# Autodesk Inventor assembly: Assembly2
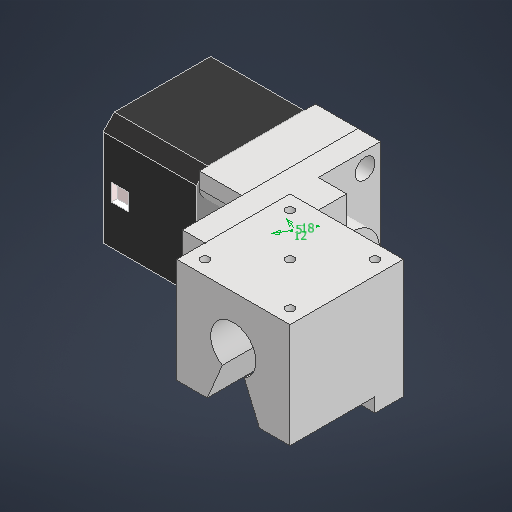
[picture p0: Inventor's stored thumbnail of the model, 512x512]
Saved by Autodesk Inventor 2025.1 (Build 291241000, 241)
## iProperties
Created: 2025-02-02
Part Number: Assembly2
Document SubType Name: Assembly
Designer: jerem
Author: jerem
## Documents named in this file (7)
- C:\Users\jerem\Documents\GitHub\Perovskite-Automated-Synthesis-System\CAD\Gantry\Assembly2.iam
- C:\Users\jerem\Documents\GitHub\Perovskite-Automated-Synthesis-System\CAD\Gantry\X Axis End.ipt
- C:\Users\jerem\Documents\GitHub\Perovskite-Automated-Synthesis-System\CAD\Non 3D Printed Parts\Motors and Servos\NEMA17 Stepper Motor.ipt
- C:\Users\jerem\Documents\GitHub\Perovskite-Automated-Synthesis-System\CAD\Gantry\end motor holder.ipt
- C:\Users\jerem\Documents\GitHub\Perovskite-Automated-Synthesis-System\CAD\Non 3D Printed Parts\Idler.ipt
- C:\Users\jerem\Documents\GitHub\Perovskite-Automated-Synthesis-System\CAD\Non 3D Printed Parts\Rod Coupler.ipt
- C:\Users\jerem\Documents\GitHub\Perovskite-Automated-Synthesis-System\CAD\Gantry\MOTOR standoff.ipt
## Components (6 placed, 6 different names)
1. X Axis End:1 — Flush:1, Mate:13, Mate:14
2. NEMA17 Stepper Motor:1 — Mate:1, Mate:2, Mate:5, Mate:6, Mate:8, Mate:10, Mate:11, Mate:12
3. end motor holder:1 — Mate:1, Mate:2, Flush:1, Mate:13, Mate:14, Mate:15
4. Idler:1 — Mate:5, Mate:6, Mate:9
5. Rod Coupler:1 — Mate:8, Mate:9
6. MOTOR standoff:1 — Mate:10, Mate:11, Mate:12, Mate:15
## Relationships (13: Mate 12, Flush 1)
- Mate:1: NEMA17 Stepper Motor:1 ↔ end motor holder:1
- Mate:2: NEMA17 Stepper Motor:1 ↔ end motor holder:1
- Flush:1: X Axis End:1 ↔ end motor holder:1
- Mate:5: NEMA17 Stepper Motor:1 ↔ Idler:1
- Mate:6: NEMA17 Stepper Motor:1 ↔ Idler:1
- Mate:8: NEMA17 Stepper Motor:1 ↔ Rod Coupler:1
- Mate:9: Idler:1 ↔ Rod Coupler:1
- Mate:10: NEMA17 Stepper Motor:1 ↔ MOTOR standoff:1
- Mate:11: NEMA17 Stepper Motor:1 ↔ MOTOR standoff:1
- Mate:12: NEMA17 Stepper Motor:1 ↔ MOTOR standoff:1
- Mate:13: X Axis End:1 ↔ end motor holder:1
- Mate:14: X Axis End:1 ↔ end motor holder:1
- Mate:15: end motor holder:1 ↔ MOTOR standoff:1
